# Autodesk Inventor assembly: test_uniones_ensamble
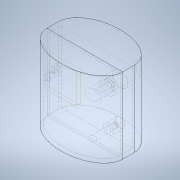
[picture p0: Inventor's stored thumbnail of the model, 180x180]
Saved by Autodesk Inventor 2021 (Build 250183000, 183)
## iProperties
Created: 2023-08-20
Part Number: test_uniones_ensamble
Document SubType Name: Assembly
Designer: Sergio
Author: Sergio
## Documents named in this file (3)
- D:\Sergio\OneDrive - Escuela Superior Politécnica del Litoral\Documentos\12vo Semestre (último)\Diseño Mecatrónico\Proyecto\Diseño Mecánico\solucion GANADORA\test_uniones_ensamble.iam
- D:\Sergio\OneDrive - Escuela Superior Politécnica del Litoral\Documentos\12vo Semestre (último)\Diseño Mecatrónico\Proyecto\Diseño Mecánico\solucion GANADORA\test\base_snap_test_down.ipt
- D:\Sergio\OneDrive - Escuela Superior Politécnica del Litoral\Documentos\12vo Semestre (último)\Diseño Mecatrónico\Proyecto\Diseño Mecánico\solucion GANADORA\test\base_snap_test_top.ipt
## Components (2 placed, 2 different names)
1. base_snap_test_down:1 — Coincidencia:1, Coincidencia:2, Coincidencia:3
2. base_snap_test_top:1 — Coincidencia:1, Coincidencia:2, Coincidencia:3
## Relationships (3: Mate 3)
- Coincidencia:1 [Mate]: base_snap_test_down:1 ↔ base_snap_test_top:1
- Coincidencia:2 [Mate]: base_snap_test_down:1 ↔ base_snap_test_top:1
- Coincidencia:3 [Mate]: base_snap_test_down:1 ↔ base_snap_test_top:1
